# Autodesk Inventor assembly: Assembly1
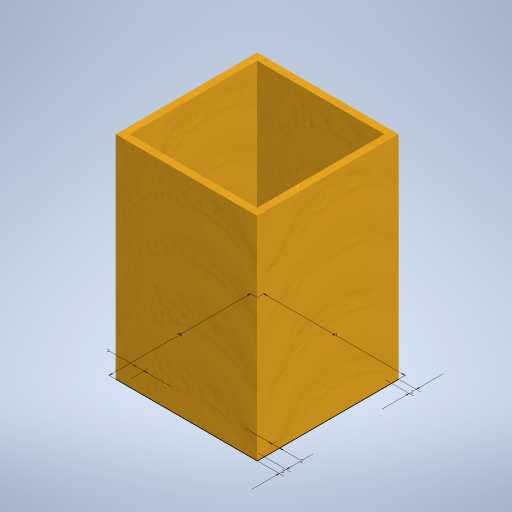
[picture p0: Inventor's stored thumbnail of the model, 512x512]
Saved by Autodesk Inventor 2024 (Build 280153000, 153)
## iProperties
Created: 2024-05-08
Part Number: Assembly1
Document SubType Name: Assembly
Designer: kamil
Author: kamil
## Documents named in this file (3)
- D:\Projects\Robotics\Linefollower_competition_gate\Assembly1.iam
- D:\Projects\Robotics\Linefollower_competition_gate\XIAO-ESP32S3 v2\XIAO-ESP32S3 v2.ipt
- D:\Projects\Robotics\Linefollower_competition_gate\sensor_block.ipt
## Components (2 placed, 2 different names)
1. XIAO-ESP32S3 v2:1 — Mate:1, Mate:2, Mate:3
2. sensor_block:1 — Mate:1, Mate:2, Mate:3
## Relationships (3: Mate 3)
- Mate:1: XIAO-ESP32S3 v2:1 ↔ sensor_block:1
- Mate:2: XIAO-ESP32S3 v2:1 ↔ sensor_block:1
- Mate:3: XIAO-ESP32S3 v2:1 ↔ sensor_block:1
